# Autodesk Inventor assembly: Osnova
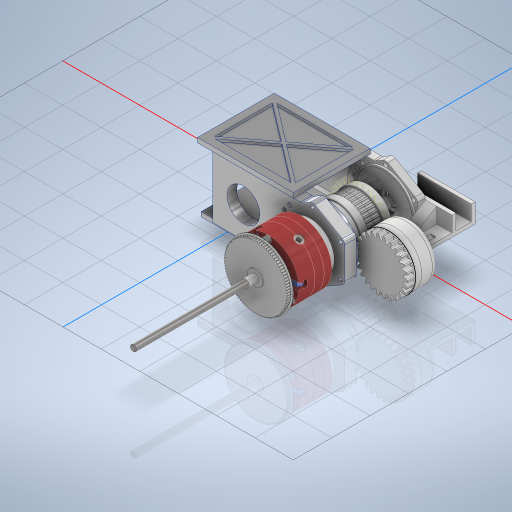
[picture p0: Inventor's stored thumbnail of the model, 512x512]
Saved by Autodesk Inventor 2024 (Build 280153000, 153)
## iProperties
Created: 2023-08-21
Part Number: Osnova
Document SubType Name: Assembly
Designer: KirikDK
Mass: 35023.4 g
Surface Area: 34965 cm^2
Volume: 16941.4 cm^3
Density: 2.06732 g/cm^3
Author: KirikDK
## Documents named in this file (17)
- C:\WorkProject\CNC_Lathe\MiniTocatka\SpindleBlock.iam
- C:\WorkProject\CNC_Lathe\MiniTocatka\PatronDerzavka.ipt
- C:\WorkProject\CNC_Lathe\MiniTocatka\SELF CENTERING CHUCK.iam
- C:\WorkProject\CNC_Lathe\MiniTocatka\ZadKriska.ipt
- C:\WorkProject\CNC_Lathe\MiniTocatka\BigPodsipnik.ipt
- C:\WorkProject\CNC_Lathe\MiniTocatka\OnPatronFlanech.ipt
- C:\WorkProject\CNC_Lathe\MiniTocatka\MuftaRemen.ipt
- C:\WorkProject\CNC_Lathe\MiniTocatka\MiniPodsipnikNatag.ipt
- C:\WorkProject\CNC_Lathe\MiniTocatka\MiniPod.ipt
- C:\WorkProject\CNC_Lathe\MiniTocatka\InstrumentalBaraban.ipt
- C:\WorkProject\CNC_Lathe\MiniTocatka\Val340.ipt
- C:\WorkProject\CNC_Lathe\MiniTocatka\PlasticZasita.ipt
- C:\WorkProject\CNC_Lathe\MiniTocatka\planeDerzavki.ipt
- C:\WorkProject\CNC_Lathe\MiniTocatka\GiroMotorKrepl.ipt
- C:\WorkProject\CNC_Lathe\MiniTocatka\ZubkataiaBig.ipt
- C:\WorkProject\CNC_Lathe\MiniTocatka\GiroMotor.ipt
- C:\WorkProject\CNC_Lathe\MiniTocatka\OnGiroGear.ipt
## Components (19 placed, 16 different names)
1. PatronDerzavka:1 — Mate:59, Mate:61, Mate:63, Mate:64, Mate:66, Mate:68, Mate:140, Flush:57, Mate:141, Mate:142, Flush:58, Mate:228
2. SELF CENTERING CHUCK:1 [sub-assembly] — Mate:59, Mate:61, Mate:134, Mate:226, Mate:227
3. ZadKriska:1 — Mate:75, Mate:76, Mate:114, Mate:130, Mate:131, Mate:147, Mate:148, Flush:59, Mate:229
4. BigPodsipnik:1 — Mate:63, Mate:64, Mate:65, Mate:67
5. OnPatronFlanech:1 — Mate:65, Mate:66
6. OnPatronFlanech:3 — Mate:67, Mate:68, Mate:69, Mate:70
7. MuftaRemen:1 — Mate:69, Mate:70, Mate:71, Mate:72
8. MuftaRemen:2 — Mate:71, Mate:72, Mate:77, Mate:78, Mate:149, Mate:150
9. MiniPod:1 — Mate:75, Mate:76, Mate:105
10. MiniPodsipnikNatag:2 — Mate:77, Mate:78, Mate:105, Mate:114
11. Val340:1 — Mate:134
12. PlasticZasita:1 — Mate:140, Flush:57, Mate:141
13. planeDerzavki:1 — Mate:142, Flush:58, Flush:60
14. GiroMotorKrepl:1 — Mate:147, Mate:148
15. ZubkataiaBig:1 — Mate:149, Mate:150
16. GiroMotor:1 — Mate:152, Mate:153
17. OnGiroGear:1 — Mate:152, Mate:153
18. InstrumentalBaraban:4 — Mate:226, Mate:227
19. planeDerzavki:2 — Mate:228, Flush:59, Mate:229, Flush:60
## Relationships (38: Mate 34, Flush 4)
- Mate:59: PatronDerzavka:1 ↔ SELF CENTERING CHUCK:1
- Mate:61: PatronDerzavka:1 ↔ SELF CENTERING CHUCK:1
- Mate:63: PatronDerzavka:1 ↔ BigPodsipnik:1
- Mate:64: PatronDerzavka:1 ↔ BigPodsipnik:1
- Mate:65: BigPodsipnik:1 ↔ OnPatronFlanech:1
- Mate:66: PatronDerzavka:1 ↔ OnPatronFlanech:1
- Mate:67: BigPodsipnik:1 ↔ OnPatronFlanech:3
- Mate:68: PatronDerzavka:1 ↔ OnPatronFlanech:3
- Mate:69: OnPatronFlanech:3 ↔ MuftaRemen:1
- Mate:70: OnPatronFlanech:3 ↔ MuftaRemen:1
- Mate:71: MuftaRemen:1 ↔ MuftaRemen:2
- Mate:72: MuftaRemen:1 ↔ MuftaRemen:2
- Mate:75: ZadKriska:1 ↔ MiniPod:1
- Mate:76: ZadKriska:1 ↔ MiniPod:1
- Mate:77: MuftaRemen:2 ↔ MiniPodsipnikNatag:2
- Mate:78: MuftaRemen:2 ↔ MiniPodsipnikNatag:2
- Mate:105: MiniPod:1 ↔ MiniPodsipnikNatag:2
- Mate:114: ZadKriska:1 ↔ MiniPodsipnikNatag:2
- Mate:130: ZadKriska:1
- Mate:131: ZadKriska:1
- Mate:134: SELF CENTERING CHUCK:1 ↔ Val340:1
- Mate:140: PatronDerzavka:1 ↔ PlasticZasita:1
- Flush:57: PatronDerzavka:1 ↔ PlasticZasita:1
- Mate:141: PatronDerzavka:1 ↔ PlasticZasita:1
- Mate:142: PatronDerzavka:1 ↔ planeDerzavki:1
- Flush:58: PatronDerzavka:1 ↔ planeDerzavki:1
- Mate:147: ZadKriska:1 ↔ GiroMotorKrepl:1
- Mate:148: ZadKriska:1 ↔ GiroMotorKrepl:1
- Mate:149: MuftaRemen:2 ↔ ZubkataiaBig:1
- Mate:150: MuftaRemen:2 ↔ ZubkataiaBig:1
- Mate:152: GiroMotor:1 ↔ OnGiroGear:1
- Mate:153: GiroMotor:1 ↔ OnGiroGear:1
- Mate:226: SELF CENTERING CHUCK:1 ↔ InstrumentalBaraban:4
- Mate:227: SELF CENTERING CHUCK:1 ↔ InstrumentalBaraban:4
- Mate:228: PatronDerzavka:1 ↔ planeDerzavki:2
- Flush:59: ZadKriska:1 ↔ planeDerzavki:2
- Mate:229: ZadKriska:1 ↔ planeDerzavki:2
- Flush:60: planeDerzavki:1 ↔ planeDerzavki:2
